# Autodesk Inventor assembly: primary-engineer-bench
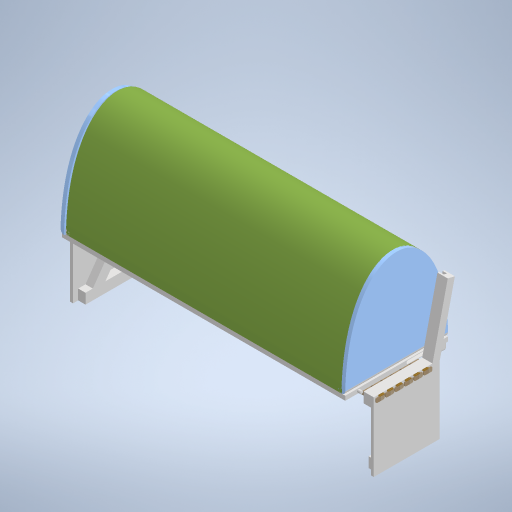
[picture p0: Inventor's stored thumbnail of the model, 512x512]
Saved by Autodesk Inventor 2023 (Build 270158030, 158C)
## iProperties
Created: 2024-09-09
Part Number: primary-engineer-bench
Document SubType Name: Assembly
Designer: Imogen Heard
d45: 13.00 deg
d44: -90.00 deg
d42: 0.000 mm
d76: 0.00 deg
d77: -90.00 deg
d73: -90.00 deg
d72: 0.00 deg
d70: 0.000 mm
backrest: -90.00 deg
sideflapA: 0.00 deg
sideflapBmm: 0.000 mm
sideflapBDEG: -0.00 deg
Author: Imogen Heard
## Documents named in this file (9)
- C:\Users\dheard\Documents\0004-inventor\3D-CAD-main\primary-engineer-bench\primary-engineer-bench.iam
- C:\Users\dheard\Documents\0004-inventor\3D-CAD-main\primary-engineer-bench\bench-end-peice.ipt
- C:\Users\dheard\Documents\0004-inventor\3D-CAD-main\primary-engineer-bench\bench-slats.ipt
- C:\Users\dheard\Documents\0004-inventor\3D-CAD-main\primary-engineer-bench\bench-end-peice_MIR.ipt
- C:\Users\dheard\Documents\0004-inventor\3D-CAD-main\primary-engineer-bench\flip-up-side.ipt
- C:\Users\dheard\Documents\0004-inventor\3D-CAD-main\primary-engineer-bench\bed-base.ipt
- C:\Users\dheard\Documents\0004-inventor\3D-CAD-main\primary-engineer-bench\back-flaps-3.ipt
- C:\Users\dheard\Documents\0004-inventor\3D-CAD-main\primary-engineer-bench\canvas-cover-stowed-V2.ipt
- C:\Users\dheard\Documents\0004-inventor\3D-CAD-main\primary-engineer-bench\canvas-cover-deployed.ipt
## Components (9 placed, 8 different names)
1. bench-end-peice:1 — Flush:1, Symmetry:1, Flush:6, lift-side-cover, Mate:1, lift-backrest
2. bench-slats:1 — Flush:1, Symmetry:1
3. bench-end-peice_MIR:1
4. flip-up-side:1 — lift-side-cover
5. bed-base:1 — Mate:1, lift-backrest, Flush:7, Mate:2, Angle:1, Rotational:3, Rotational:4, Flush:8, Flush:9, Flush:10, Mate:3, Mate:4, Flush:11
6. back-flaps-3:1 — Rotational:3
7. back-flaps-3:2 — Rotational:4
8. canvas-cover-stowed-V2:1 — Flush:8, Flush:9, Flush:10
9. canvas-cover-deployed:1 — Mate:3, Mate:4, Flush:11
## Relationships (17: Flush 7, RevoluteJoint 4, Mate 4, Symmetry 1, Angle 1)
- Flush:1: bench-end-peice:1 ↔ bench-slats:1
- Symmetry:1: bench-end-peice:1 ↔ bench-slats:1
- Flush:6 (5 mm): bench-end-peice:1
- lift-side-cover [RevoluteJoint]: bench-end-peice:1 ↔ flip-up-side:1
- Mate:1: bench-end-peice:1 ↔ bed-base:1
- lift-backrest [RevoluteJoint]: bench-end-peice:1 ↔ bed-base:1
- Flush:7 (20 mm): bed-base:1
- Mate:2: bed-base:1
- Angle:1 (90 deg): bed-base:1
- Rotational:3 [RevoluteJoint]: bed-base:1 ↔ back-flaps-3:1
- Rotational:4 [RevoluteJoint]: bed-base:1 ↔ back-flaps-3:2
- Flush:8: bed-base:1 ↔ canvas-cover-stowed-V2:1
- Flush:9: bed-base:1 ↔ canvas-cover-stowed-V2:1
- Flush:10: bed-base:1 ↔ canvas-cover-stowed-V2:1
- Mate:3: bed-base:1 ↔ canvas-cover-deployed:1
- Mate:4: bed-base:1 ↔ canvas-cover-deployed:1
- Flush:11 (22.5 mm): bed-base:1 ↔ canvas-cover-deployed:1
